# Autodesk Inventor assembly: Ensamble_Pierna
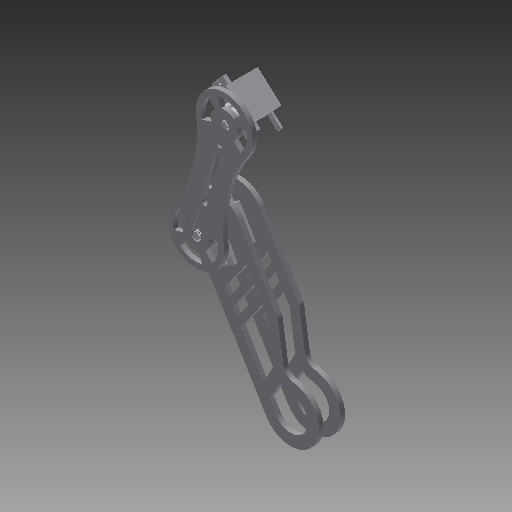
[picture p0: Inventor's stored thumbnail of the model, 512x512]
Saved by Autodesk Inventor 2019 (Build 230136000, 136)
## iProperties
Created: 2020-02-12
Part Number: Ensamble_Pierna
Document SubType Name: Assembly
Designer: jacqu
Mass: 47.369 g
Surface Area: 327.582 cm^2
Volume: 47.369 cm^3
Density: 1 g/cm^3
Author: jacqu
## Documents named in this file (4)
- E:\Escritorio\Temporal\Documentos\Robótica I\ProyectoCuadrupedo\Proyecto1\Proyecto1\Pata - Ensamble.iam
- E:\Escritorio\Temporal\Documentos\Robótica I\ProyectoCuadrupedo\Proyecto1\Proyecto1\Pata - Antebrazo.ipt
- E:\Escritorio\Temporal\Documentos\Robótica I\ProyectoCuadrupedo\Proyecto1\Proyecto1\Pata - Brazo.ipt
- E:\Escritorio\Temporal\Documentos\Robótica I\ProyectoCuadrupedo\Proyecto1\Proyecto1\Servo - Componente.ipt
## Components (5 placed, 3 different names)
1. Pata - Antebrazo:1 — Mate:13, Mate:15, Coincidencia:16, Coincidencia:17
2. Pata - Brazo:1 — Mate:1, Mate:7, Mate:8
3. Servo - Componente:1 — Mate:1, Mate:7, Mate:8, Mate:9, Mate:10, Mate:13, Nivelación:1, Coincidencia:17
4. Servo - Componente:2 — Mate:15, Coincidencia:16
5. Pata - Brazo:2 — Mate:9, Mate:10, Nivelación:1
## Relationships (10: Mate 9, Flush 1)
- Mate:1: Pata - Brazo:1 ↔ Servo - Componente:1
- Mate:7: Pata - Brazo:1 ↔ Servo - Componente:1
- Mate:8: Pata - Brazo:1 ↔ Servo - Componente:1
- Mate:9: Servo - Componente:1 ↔ Pata - Brazo:2
- Mate:10: Servo - Componente:1 ↔ Pata - Brazo:2
- Mate:13: Pata - Antebrazo:1 ↔ Servo - Componente:1
- Mate:15: Pata - Antebrazo:1 ↔ Servo - Componente:2
- Nivelación:1 [Flush]: Servo - Componente:1 ↔ Pata - Brazo:2
- Coincidencia:16 [Mate]: Pata - Antebrazo:1 ↔ Servo - Componente:2
- Coincidencia:17 [Mate]: Pata - Antebrazo:1 ↔ Servo - Componente:1
